# Autodesk Inventor assembly: 110033226_iam_03_大橋
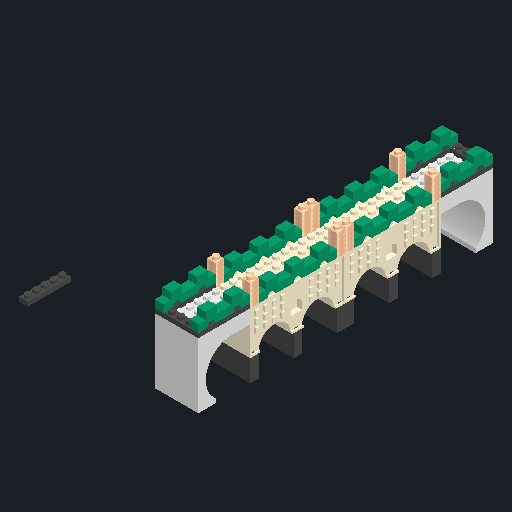
[picture p0: Inventor's stored thumbnail of the model, 512x512]
Saved by Autodesk Inventor 2022 (Build 260153000, 153)
## iProperties
Created: 2022-06-23
Part Number: 110033226_iam_03_大橋
Document SubType Name: Assembly
Designer: User
Author: User
## Documents named in this file (6)
- D:\D-disk\pomelo\大一\下學期\機械設計製圖\1100332260_LEGOproj_沒有公主城堡\110033226_iam_03_大橋.iam
- D:\D-disk\pomelo\大一\下學期\機械設計製圖\1100332260_LEGOproj_沒有公主城堡\110033226_ipt_17_大橋.ipt
- D:\D-disk\pomelo\大一\下學期\機械設計製圖\1100332260_LEGOproj_沒有公主城堡\110033226_ipt_18_大橋圍牆.ipt
- D:\D-disk\pomelo\大一\下學期\機械設計製圖\1100332260_LEGOproj_沒有公主城堡\110033226_ipt_06_磚塊樺木(1x1).ipt
- D:\D-disk\pomelo\大一\下學期\機械設計製圖\1100332260_LEGOproj_沒有公主城堡\110033226_ipt_16_圍牆.ipt
- D:\D-disk\pomelo\大一\下學期\機械設計製圖\1100332260_LEGOproj_沒有公主城堡\110033226_ipt_19_大橋接通道路.ipt
## Components (101 placed, 5 different names)
1. 110033226_ipt_19_大橋接通道路:1 — 貼合:10, 貼合:11, 貼合:12, 貼合:16, 貼合:17, 貼合:18, 貼合:21, 貼合:22, 貼合:23, 貼合:27, 貼合:28, 貼合:29
2. 110033226_ipt_19_大橋接通道路:2 — 貼合:13, 貼合:14, 貼合:15
3. 110033226_ipt_16_圍牆:34 — 貼合:16, 貼合:17, 貼合:18, 貼合:19, 貼合:20, 貼合:24, 貼合:25
4. 110033226_ipt_16_圍牆:35 — 貼合:27, 貼合:28, 貼合:29
5. 110033226_ipt_16_圍牆:36 — 貼合:21, 貼合:22, 貼合:23, 貼合:26
6. 110033226_ipt_16_圍牆:37
7. 110033226_ipt_16_圍牆:38 — 貼合:30, 貼合:31, 貼合:33, 貼合:34
8. 110033226_ipt_16_圍牆:39
9. 110033226_ipt_16_圍牆:40 — 貼合:32
10. 110033226_ipt_17_大橋:1 — 貼合:1, 貼合:2, 貼合:3, 貼合:4, 貼合:5, 貼合:7, 貼合:8, 貼合:9, 貼合:10, 貼合:12
11. 110033226_ipt_17_大橋:2 — 貼合:13, 貼合:14, 貼合:15
12. 110033226_ipt_18_大橋圍牆:14 — 貼合:24, 貼合:25, 貼合:26
13. 110033226_ipt_18_大橋圍牆:13 — 貼合:19, 貼合:20
14. 110033226_ipt_18_大橋圍牆:15
15. 110033226_ipt_18_大橋圍牆:16
16. 110033226_ipt_18_大橋圍牆:17 — 貼合:32, 貼合:33, 貼合:34
17. 110033226_ipt_18_大橋圍牆:18 — 貼合:30, 貼合:31
18. 110033226_ipt_18_大橋圍牆:19
19. 110033226_ipt_18_大橋圍牆:20
20. 110033226_ipt_18_大橋圍牆:1 — 貼合:1, 貼合:2, 貼合:3, 貼合:6
21. 110033226_ipt_18_大橋圍牆:2
22. 110033226_ipt_18_大橋圍牆:3
23. 110033226_ipt_18_大橋圍牆:4
24. 110033226_ipt_18_大橋圍牆:5
25. 110033226_ipt_18_大橋圍牆:6
26. 110033226_ipt_18_大橋圍牆:7
27. 110033226_ipt_18_大橋圍牆:8
28. 110033226_ipt_18_大橋圍牆:9
29. 110033226_ipt_18_大橋圍牆:10
30. 110033226_ipt_18_大橋圍牆:11
31. 110033226_ipt_18_大橋圍牆:12
32. 110033226_ipt_06_磚塊樺木(1x1):1 — 貼合:4, 貼合:5, 貼合:6, 貼合:11
33. 110033226_ipt_06_磚塊樺木(1x1):5
34. 110033226_ipt_06_磚塊樺木(1x1):6
35. 110033226_ipt_06_磚塊樺木(1x1):7
36. 110033226_ipt_06_磚塊樺木(1x1):8
37. 110033226_ipt_06_磚塊樺木(1x1):9
38. 110033226_ipt_06_磚塊樺木(1x1):10
39. 110033226_ipt_06_磚塊樺木(1x1):11
40. 110033226_ipt_06_磚塊樺木(1x1):12
41. 110033226_ipt_06_磚塊樺木(1x1):13
42. 110033226_ipt_06_磚塊樺木(1x1):14
43. 110033226_ipt_06_磚塊樺木(1x1):15
44. 110033226_ipt_06_磚塊樺木(1x1):16
45. 110033226_ipt_06_磚塊樺木(1x1):17
46. 110033226_ipt_06_磚塊樺木(1x1):18
47. 110033226_ipt_06_磚塊樺木(1x1):19
48. 110033226_ipt_06_磚塊樺木(1x1):20
49. 110033226_ipt_06_磚塊樺木(1x1):21
50. 110033226_ipt_06_磚塊樺木(1x1):22
51. 110033226_ipt_06_磚塊樺木(1x1):23
52. 110033226_ipt_16_圍牆:2 — 貼合:7, 貼合:8, 貼合:9
53. 110033226_ipt_16_圍牆:5
54. 110033226_ipt_16_圍牆:6
55. 110033226_ipt_16_圍牆:7
56. 110033226_ipt_16_圍牆:8
57. 110033226_ipt_16_圍牆:9
58. 110033226_ipt_16_圍牆:10
59. 110033226_ipt_16_圍牆:11
60. 110033226_ipt_16_圍牆:12
61. 110033226_ipt_16_圍牆:13
62. 110033226_ipt_16_圍牆:14
63. 110033226_ipt_16_圍牆:15
64. 110033226_ipt_16_圍牆:16
65. 110033226_ipt_16_圍牆:17
66. 110033226_ipt_16_圍牆:18
67. 110033226_ipt_06_磚塊樺木(1x1):24
68. 110033226_ipt_06_磚塊樺木(1x1):25
69. 110033226_ipt_06_磚塊樺木(1x1):26
70. 110033226_ipt_06_磚塊樺木(1x1):27
71. 110033226_ipt_06_磚塊樺木(1x1):28
72. 110033226_ipt_06_磚塊樺木(1x1):29
73. 110033226_ipt_06_磚塊樺木(1x1):30
74. 110033226_ipt_06_磚塊樺木(1x1):31
75. 110033226_ipt_06_磚塊樺木(1x1):32
76. 110033226_ipt_06_磚塊樺木(1x1):33
77. 110033226_ipt_06_磚塊樺木(1x1):34
78. 110033226_ipt_06_磚塊樺木(1x1):35
79. 110033226_ipt_06_磚塊樺木(1x1):36
80. 110033226_ipt_06_磚塊樺木(1x1):37
81. 110033226_ipt_06_磚塊樺木(1x1):38
82. 110033226_ipt_06_磚塊樺木(1x1):39
83. 110033226_ipt_06_磚塊樺木(1x1):40
84. 110033226_ipt_06_磚塊樺木(1x1):41
85. 110033226_ipt_06_磚塊樺木(1x1):42
86. 110033226_ipt_06_磚塊樺木(1x1):43
87. 110033226_ipt_16_圍牆:19
88. 110033226_ipt_16_圍牆:20
89. 110033226_ipt_16_圍牆:21
90. 110033226_ipt_16_圍牆:22
91. 110033226_ipt_16_圍牆:23
92. 110033226_ipt_16_圍牆:24
93. 110033226_ipt_16_圍牆:25
94. 110033226_ipt_16_圍牆:26
95. 110033226_ipt_16_圍牆:27
96. 110033226_ipt_16_圍牆:28
97. 110033226_ipt_16_圍牆:29
98. 110033226_ipt_16_圍牆:30
99. 110033226_ipt_16_圍牆:31
100. 110033226_ipt_16_圍牆:32
101. 110033226_ipt_16_圍牆:33
## Component patterns: (2 elements, first: 110033226_ipt_17_大橋:1), (2 elements, first: 110033226_ipt_18_大橋圍牆:14 + 110033226_ipt_18_大橋圍牆:13), (2 elements, first: 110033226_ipt_18_大橋圍牆:17 + 110033226_ipt_18_大橋圍牆:18), (4 elements), (6 elements, first: 110033226_ipt_18_大橋圍牆:1), (3 elements), 元件陣列 3:2 (4 elements), 元件陣列 1:2 (6 elements), 元件陣列 7:2 (3 elements), (5 elements, first: 110033226_ipt_06_磚塊樺木(1x1):1), 元件陣列 2:2 (5 elements), 元件陣列 2:3 (5 elements), 元件陣列 2:4 (5 elements), (5 elements, first: 110033226_ipt_16_圍牆:2), 元件陣列 6:2 (5 elements), 元件陣列 6:3 (5 elements), 元件陣列 2:5 (5 elements), 元件陣列 2:6 (5 elements), 元件陣列 2:7 (5 elements), 元件陣列 2:8 (5 elements), 元件陣列 6:4 (5 elements), 元件陣列 6:5 (5 elements), 元件陣列 6:6 (5 elements)
## Relationships (34: Mate 34)
- 貼合:1 [Mate]: 110033226_ipt_17_大橋:1 ↔ 110033226_ipt_18_大橋圍牆:1
- 貼合:2 [Mate]: 110033226_ipt_17_大橋:1 ↔ 110033226_ipt_18_大橋圍牆:1
- 貼合:3 [Mate]: 110033226_ipt_17_大橋:1 ↔ 110033226_ipt_18_大橋圍牆:1
- 貼合:4 [Mate]: 110033226_ipt_17_大橋:1 ↔ 110033226_ipt_06_磚塊樺木(1x1):1
- 貼合:5 [Mate]: 110033226_ipt_17_大橋:1 ↔ 110033226_ipt_06_磚塊樺木(1x1):1
- 貼合:6 [Mate]: 110033226_ipt_18_大橋圍牆:1 ↔ 110033226_ipt_06_磚塊樺木(1x1):1
- 貼合:7 [Mate]: 110033226_ipt_17_大橋:1 ↔ 110033226_ipt_16_圍牆:2
- 貼合:8 [Mate]: 110033226_ipt_17_大橋:1 ↔ 110033226_ipt_16_圍牆:2
- 貼合:9 [Mate]: 110033226_ipt_17_大橋:1 ↔ 110033226_ipt_16_圍牆:2
- 貼合:10 [Mate]: 110033226_ipt_19_大橋接通道路:1 ↔ 110033226_ipt_17_大橋:1
- 貼合:11 [Mate]: 110033226_ipt_19_大橋接通道路:1 ↔ 110033226_ipt_06_磚塊樺木(1x1):1
- 貼合:12 [Mate]: 110033226_ipt_19_大橋接通道路:1 ↔ 110033226_ipt_17_大橋:1
- 貼合:13 [Mate]: 110033226_ipt_19_大橋接通道路:2 ↔ 110033226_ipt_17_大橋:2
- 貼合:14 [Mate]: 110033226_ipt_19_大橋接通道路:2 ↔ 110033226_ipt_17_大橋:2
- 貼合:15 [Mate]: 110033226_ipt_19_大橋接通道路:2 ↔ 110033226_ipt_17_大橋:2
- 貼合:16 [Mate]: 110033226_ipt_19_大橋接通道路:1 ↔ 110033226_ipt_16_圍牆:34
- 貼合:17 [Mate]: 110033226_ipt_19_大橋接通道路:1 ↔ 110033226_ipt_16_圍牆:34
- 貼合:18 [Mate]: 110033226_ipt_19_大橋接通道路:1 ↔ 110033226_ipt_16_圍牆:34
- 貼合:19 [Mate]: 110033226_ipt_16_圍牆:34 ↔ 110033226_ipt_18_大橋圍牆:13
- 貼合:20 [Mate]: 110033226_ipt_16_圍牆:34 ↔ 110033226_ipt_18_大橋圍牆:13
- 貼合:21 [Mate]: 110033226_ipt_19_大橋接通道路:1 ↔ 110033226_ipt_16_圍牆:36
- 貼合:22 [Mate]: 110033226_ipt_19_大橋接通道路:1 ↔ 110033226_ipt_16_圍牆:36
- 貼合:23 [Mate]: 110033226_ipt_19_大橋接通道路:1 ↔ 110033226_ipt_16_圍牆:36
- 貼合:24 [Mate]: 110033226_ipt_16_圍牆:34 ↔ 110033226_ipt_18_大橋圍牆:14
- 貼合:25 [Mate]: 110033226_ipt_16_圍牆:34 ↔ 110033226_ipt_18_大橋圍牆:14
- 貼合:26 [Mate]: 110033226_ipt_16_圍牆:36 ↔ 110033226_ipt_18_大橋圍牆:14
- 貼合:27 [Mate]: 110033226_ipt_19_大橋接通道路:1 ↔ 110033226_ipt_16_圍牆:35
- 貼合:28 [Mate]: 110033226_ipt_19_大橋接通道路:1 ↔ 110033226_ipt_16_圍牆:35
- 貼合:29 [Mate]: 110033226_ipt_19_大橋接通道路:1 ↔ 110033226_ipt_16_圍牆:35
- 貼合:30 [Mate]: 110033226_ipt_16_圍牆:38 ↔ 110033226_ipt_18_大橋圍牆:18
- 貼合:31 [Mate]: 110033226_ipt_16_圍牆:38 ↔ 110033226_ipt_18_大橋圍牆:18
- 貼合:32 [Mate]: 110033226_ipt_16_圍牆:40 ↔ 110033226_ipt_18_大橋圍牆:17
- 貼合:33 [Mate]: 110033226_ipt_16_圍牆:38 ↔ 110033226_ipt_18_大橋圍牆:17
- 貼合:34 [Mate]: 110033226_ipt_16_圍牆:38 ↔ 110033226_ipt_18_大橋圍牆:17
